# Autodesk Inventor assembly: ASY PNS-0110 frame left floor
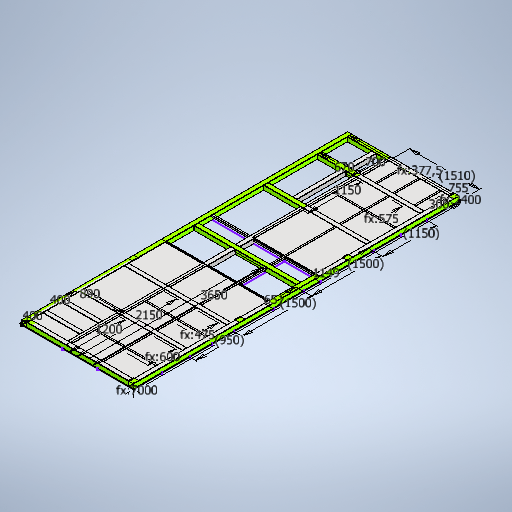
[picture p0: Inventor's stored thumbnail of the model, 512x512]
Saved by Autodesk Inventor 2025 (Build 290162010, 162A)
## iProperties
Created: 2025-03-10
Part Number: ASY PNS-0110 frame left floor
Document SubType Name: Assembly
Designer: admin
_SolveAssemblyDoc: Frame Generator Solve Assembly
_Version: 25.0.0
Author: admin
## Documents named in this file (7)
- C:\Users\admin\YandexDisk-badmisterfox\home pc\Inventor\PNS-Panaevsk\ASY PNS-0110 frame left floor.iam
- C:\Users\admin\YandexDisk-badmisterfox\home pc\Inventor\PNS-Panaevsk\PNS-0110 frame left floor.ipt
- C:\Users\admin\YandexDisk-badmisterfox\home pc\Inventor\PNS-Panaevsk\ASY PNS-0110 frame left floor\Frame\Frame 1741580713954.iam
- C:\Users\admin\YandexDisk-badmisterfox\home pc\Inventor\PNS-Panaevsk\PNS-0111 floor sheet 1.ipt
- C:\Users\admin\YandexDisk-badmisterfox\home pc\Inventor\PNS-Panaevsk\PNS-0111 floor sheet 2.ipt
- C:\Users\admin\YandexDisk-badmisterfox\home pc\Inventor\PNS-Panaevsk\PNS-0113 floor sheet 3.ipt
- C:\Users\admin\YandexDisk-badmisterfox\home pc\Inventor\PNS-Panaevsk\PNS-0114 floor sheet 4.ipt
## Components (6 placed, 6 different names)
1. PNS-0110 frame left floor:1
2. Frame 1741580713954:1 [sub-assembly] — Rigid:1, Rigid:2, Rigid:3, Rigid:4
3. PNS-0111 floor sheet 1:1 — Rigid:1
4. PNS-0111 floor sheet 2:2 — Rigid:2
5. PNS-0113 floor sheet 3:1 — Rigid:3
6. PNS-0114 floor sheet 4:1 — Rigid:4
## Relationships (4: WeldJoint 4)
- Rigid:1 [WeldJoint]: Frame 1741580713954:1 ↔ PNS-0111 floor sheet 1:1
- Rigid:2 [WeldJoint] (-116 mm): Frame 1741580713954:1 ↔ PNS-0111 floor sheet 2:2
- Rigid:3 [WeldJoint] (-116 mm): Frame 1741580713954:1 ↔ PNS-0113 floor sheet 3:1
- Rigid:4 [WeldJoint] (-116 mm): Frame 1741580713954:1 ↔ PNS-0114 floor sheet 4:1
